# Autodesk Inventor assembly: Main_v6
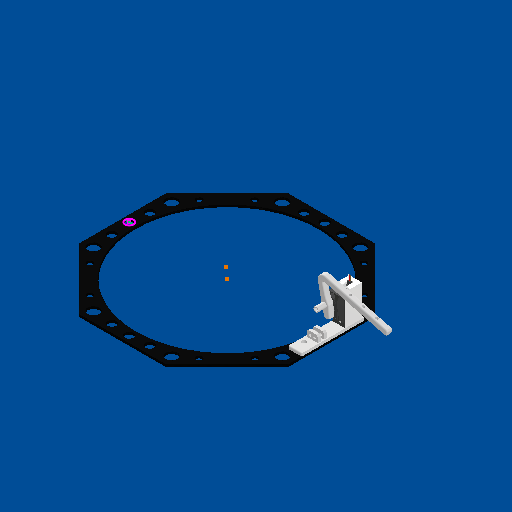
[picture p0: Inventor's stored thumbnail of the model, 512x512]
Saved by Autodesk Inventor 2026.2 (Build 302298000, 298)
## iProperties
Created: 2026-03-12
Part Number: Main_v6
Document SubType Name: Assembly
Designer: Thoma
Author: Thoma
## Documents named in this file (6)
- C:\Users\Thoma\OneDrive\Desktop\dir\telescope_cover\main\version_2\Main_v6.iam
- C:\Users\Thoma\OneDrive\Desktop\dir\telescope_cover\telescope\version_4\Telescope_End.ipt
- C:\Users\Thoma\OneDrive\Desktop\dir\telescope_cover\cover\base_plate_v18.ipt
- C:\Users\Thoma\OneDrive\Desktop\dir\telescope_cover\servo\DSS-M15S Servo.ipt
- C:\Users\Thoma\OneDrive\Desktop\dir\telescope_cover\cover\rod_v13.ipt
- C:\Users\Thoma\OneDrive\Desktop\dir\telescope_cover\cover\servo_attach_derive.ipt
## Components (5 placed, 5 different names)
1. Telescope_End:1 — Mate:1, Angle:1, Mate:2
2. base_plate_v18:1 — Mate:1, Angle:1, Mate:2, Mate:4, Mate:5, Mate:6
3. DSS-M15S Servo:1 — Mate:4, Mate:5, Mate:6, Mate:7, Mate:8
4. rod_v13:1 — Mate:9, Mate:10, Angle:2
5. servo_attach_derive:1 — Mate:7, Mate:8, Mate:9, Mate:10, Angle:2
## Relationships (11: Mate 9, Angle 2)
- Mate:1: Telescope_End:1 ↔ base_plate_v18:1
- Angle:1 (0 deg): Telescope_End:1 ↔ base_plate_v18:1
- Mate:2: Telescope_End:1 ↔ base_plate_v18:1
- Mate:4 (0.5 mm): base_plate_v18:1 ↔ DSS-M15S Servo:1
- Mate:5 (0.5 mm): base_plate_v18:1 ↔ DSS-M15S Servo:1
- Mate:6: base_plate_v18:1 ↔ DSS-M15S Servo:1
- Mate:7: DSS-M15S Servo:1 ↔ servo_attach_derive:1
- Mate:8: DSS-M15S Servo:1 ↔ servo_attach_derive:1
- Mate:9: rod_v13:1 ↔ servo_attach_derive:1
- Mate:10: rod_v13:1 ↔ servo_attach_derive:1
- Angle:2 (0 deg): rod_v13:1 ↔ servo_attach_derive:1
